# Autodesk Inventor assembly: MX-106T+idle.ipt
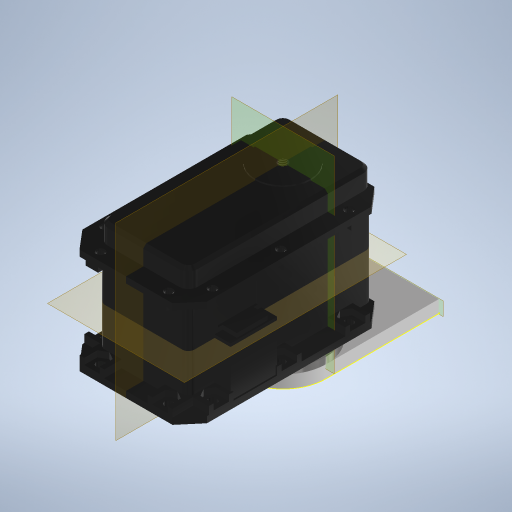
[picture p0: Inventor's stored thumbnail of the model, 512x512]
Saved by Autodesk Inventor 2024.3 (Build 283343000, 343)
## iProperties
Created: 2022-08-09
Part Number: MX-106T+idle.ipt
Document SubType Name: Assembly
Designer: 박지훈
Author: 박지훈
## Documents named in this file (5)
- C:\Users\gretc\Desktop\inventor_part\다이나믹셀\MX-106T+idle.ipt.iam
- C:\Users\gretc\Desktop\inventor_part\아이들러\64아이들러.iam
- C:\Users\gretc\Desktop\inventor_part\다이나믹셀\MX-106T.ipt
- C:\Users\gretc\Desktop\inventor_part\foot_.ipt
- C:\Users\gretc\Desktop\inventor_part\robot_FOOT.ipt
## Components (4 placed, 4 different names)
1. 64아이들러:1 [sub-assembly] — 삽입:1, 플러쉬:1
2. MX-106T:1 — 삽입:1
3. foot_:1 — 플러쉬:1, 플러쉬:3, 플러쉬:4
4. robot_FOOT:1 — 플러쉬:3, 플러쉬:4
## Relationships (4: Flush 3, Insert 1)
- 삽입:1 [Insert] (0.06 mm): 64아이들러:1 ↔ MX-106T:1
- 플러쉬:1 [Flush]: 64아이들러:1 ↔ foot_:1
- 플러쉬:3 [Flush]: foot_:1 ↔ robot_FOOT:1
- 플러쉬:4 [Flush]: foot_:1 ↔ robot_FOOT:1
